# Autodesk Inventor assembly: AxisZ
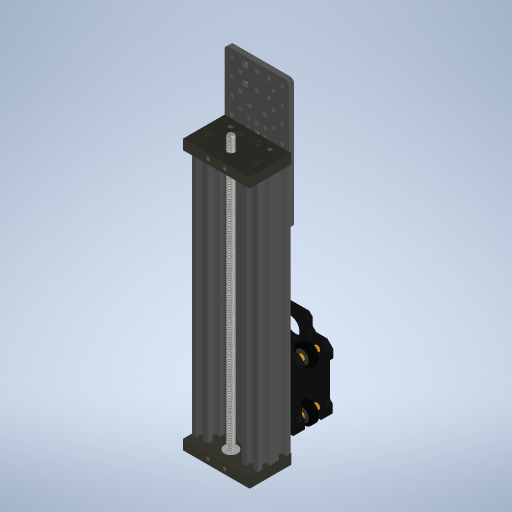
[picture p0: Inventor's stored thumbnail of the model, 512x512]
Saved by Autodesk Inventor 2024.3 (Build 283343000, 343)
## iProperties
Created: 2024-08-27
Part Number: AxisZ
Document SubType Name: Assembly
Designer: Admin
Author: Admin
## Documents named in this file (7)
- C:\Users\migue\Documents\GitHub\RobotCartesiano\DiseñoBrazo\Assemblies\AxisZ.iam
- C:\Users\migue\Documents\GitHub\RobotCartesiano\DiseñoBrazo\Axis\AxisZ\Structure\C-Beam4080.ipt
- C:\Users\migue\Documents\GitHub\RobotCartesiano\DiseñoBrazo\Axis\AxisZ\Structure\C-BeamEnd.ipt
- C:\Users\migue\Documents\GitHub\RobotCartesiano\DiseñoBrazo\Axis\AxisZ\Structure\Bearing8x16x5.ipt
- C:\Users\migue\Documents\GitHub\RobotCartesiano\DiseñoBrazo\Axis\AxisZ\Structure\BallScrew.ipt
- C:\Users\migue\Documents\GitHub\RobotCartesiano\DiseñoBrazo\Assemblies\SlidingHolder.iam
- C:\Users\migue\Documents\GitHub\RobotCartesiano\DiseñoBrazo\AuxiliarPieces\GantryPlate\C-Beam CNC.ipt
## Components (8 placed, 6 different names)
1. SlidingHolder:1 [sub-assembly] — Mate:9, Flush:6
2. C-Beam CNC:1 — Mate:8
3. C-Beam4080:1 — Flush:1, Mate:1, Mate:2, Flush:2, Flush:3, Flush:4, Mate:9
4. C-BeamEnd:2 — Mate:2, Flush:3, Flush:4, Mate:3, Mate:4, Flush:5, Flush:6
5. C-BeamEnd:3 — Flush:1, Mate:1, Flush:2, Mate:5, Mate:6, Mate:7, Mate:8
6. Bearing8x16x5:1 — Mate:3, Mate:4
7. Bearing8x16x5:2 — Mate:5, Mate:6
8. BallScrew:1 — Mate:7, Flush:5
## Relationships (15: Mate 9, Flush 6)
- Flush:1: C-Beam4080:1 ↔ C-BeamEnd:3
- Mate:1: C-Beam4080:1 ↔ C-BeamEnd:3
- Mate:2: C-Beam4080:1 ↔ C-BeamEnd:2
- Flush:2: C-Beam4080:1 ↔ C-BeamEnd:3
- Flush:3: C-Beam4080:1 ↔ C-BeamEnd:2
- Flush:4: C-Beam4080:1 ↔ C-BeamEnd:2
- Mate:3: C-BeamEnd:2 ↔ Bearing8x16x5:1
- Mate:4: C-BeamEnd:2 ↔ Bearing8x16x5:1
- Mate:5: C-BeamEnd:3 ↔ Bearing8x16x5:2
- Mate:6: C-BeamEnd:3 ↔ Bearing8x16x5:2
- Mate:7: C-BeamEnd:3 ↔ BallScrew:1
- Flush:5: C-BeamEnd:2 ↔ BallScrew:1
- Mate:8: C-Beam CNC:1 ↔ C-BeamEnd:3
- Mate:9 (4.9 mm): SlidingHolder:1 ↔ C-Beam4080:1
- Flush:6 (26 mm): SlidingHolder:1 ↔ C-BeamEnd:2
